# Autodesk Inventor assembly: ENSAMBLE
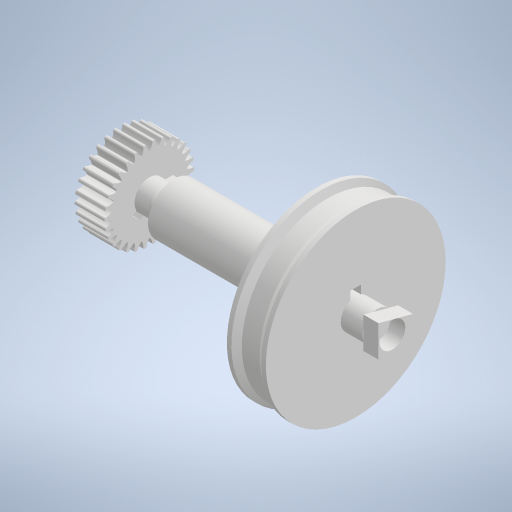
[picture p0: Inventor's stored thumbnail of the model, 512x512]
Saved by Autodesk Inventor 2024 (Build 280153000, 153)
## iProperties
Created: 2024-03-07
Part Number: ENSAMBLE
Document SubType Name: Assembly
Designer: Admin
Author: Admin
## Documents named in this file (6)
- C:\Users\Admin\Downloads\ENSAMBLE.iam
- C:\Users\Admin\Downloads\POLEA.ipt
- C:\Users\Admin\Downloads\ENGRANE.ipt
- C:\Users\Admin\Downloads\CUÑA.ipt
- C:\Users\Admin\Downloads\EJE_CUÑEROS.ipt
- C:\Users\Admin\Desktop\parte ensamble.ipt
## Components (5 placed, 5 different names)
1. POLEA:1 — Rigid:1
2. ENGRANE:1 — Rotational:1, Flush:1
3. CUÑA:1 — Planar:1, Planar:2
4. EJE_CUÑEROS:1 — Rigid:1, Rotational:1, Flush:1, Planar:1, Planar:2, Rotational:2
5. parte ensamble:1 — Rotational:2
## Relationships (6: RevoluteJoint 2, PlanarJoint 2, WeldJoint 1, Flush 1)
- Rigid:1 [WeldJoint]: POLEA:1 ↔ EJE_CUÑEROS:1
- Rotational:1 [RevoluteJoint]: ENGRANE:1 ↔ EJE_CUÑEROS:1
- Flush:1: ENGRANE:1 ↔ EJE_CUÑEROS:1
- Planar:1: CUÑA:1 ↔ EJE_CUÑEROS:1
- Planar:2: CUÑA:1 ↔ EJE_CUÑEROS:1
- Rotational:2 [RevoluteJoint]: EJE_CUÑEROS:1 ↔ parte ensamble:1
